# Autodesk Inventor assembly: linearbearing-bolted
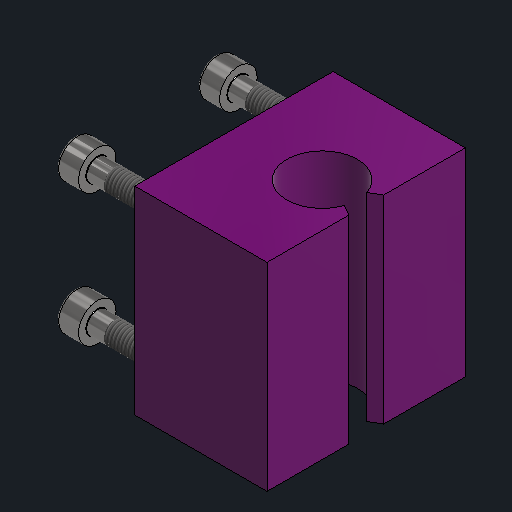
[picture p0: Inventor's stored thumbnail of the model, 512x512]
Saved by Autodesk Inventor 2027.1 (Build 311270010, 270A)
## iProperties
Part Number: linearbearing-bolted
Document SubType Name: Assembly
Designer: queezz
Author: queezz
## Documents named in this file (3)
- C:\Users\queezz\Dropbox\Drawings\pihti-cad\bellows-probe\linearbearing-bolted.iam
- C:\Users\queezz\Dropbox\Drawings\pihti-cad\bellows-probe\linearbearing.ipt
- C:\Users\queezz\Dropbox\Drawings\pihti-cad\ContentCenter\Fastners\M5x20-SHCS.ipt
## Components (5 placed, 2 different names)
1. linearbearing:1 — Rigid:3, Rigid:1, Rigid:2, Rigid:4
2. AS 1420 - Metric M5 x 20:4 — Rigid:4
3. AS 1420 - Metric M5 x 20:3 — Rigid:2
4. AS 1420 - Metric M5 x 20:2 — Rigid:1
5. AS 1420 - Metric M5 x 20:1 — Rigid:3
## Relationships (4: WeldJoint 4)
- Rigid:3 [WeldJoint] (15 mm): linearbearing:1 ↔ AS 1420 - Metric M5 x 20:1
- Rigid:1 [WeldJoint] (15 mm): linearbearing:1 ↔ AS 1420 - Metric M5 x 20:2
- Rigid:2 [WeldJoint] (15 mm): linearbearing:1 ↔ AS 1420 - Metric M5 x 20:3
- Rigid:4 [WeldJoint] (15 mm): linearbearing:1 ↔ AS 1420 - Metric M5 x 20:4
## Named parameters: d123_d93 = 15 mm, d124_d94 = -1.444006 deg, d122_d92 = 15 mm, d121_d97 = 15 mm
